# Autodesk Inventor assembly: Window_Cabinet
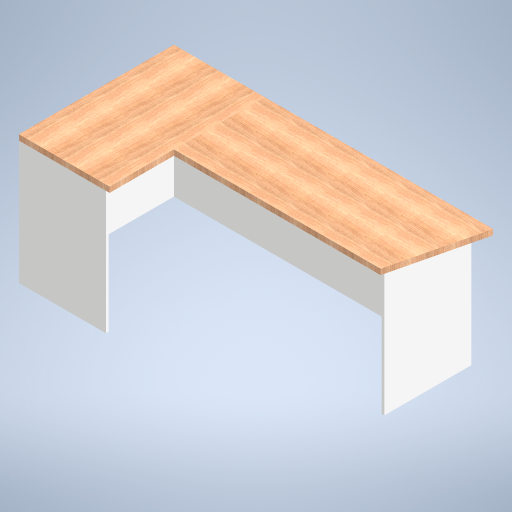
[picture p0: Inventor's stored thumbnail of the model, 512x512]
Saved by Autodesk Inventor 2024 (Build 280153000, 153)
## iProperties
Created: 2023-05-06
Part Number: Window_Cabinet
Document SubType Name: Assembly
Designer: Tom
Author: Tom
## Documents named in this file (6)
- C:\Users\Tom\Documents\Tom_Levers_Public_Git_Repository\Inventor\Mobility\Window_Cabinet\Window_Cabinet.iam
- C:\Users\Tom\Documents\Tom_Levers_Public_Git_Repository\Inventor\Mobility\Window_Cabinet\Plywood--0.75_x_34_x_88_in.ipt
- C:\Users\Tom\Documents\Tom_Levers_Public_Git_Repository\Inventor\Mobility\Window_Cabinet\Plywood--0.75_x_34_x_42_in.ipt
- C:\Users\Tom\Documents\Tom_Levers_Public_Git_Repository\Inventor\Mobility\Window_Cabinet\Plywood--0.75_x_34_x_23.25_in.ipt
- C:\Users\Tom\Documents\Tom_Levers_Public_Git_Repository\Inventor\Mobility\Window_Cabinet\Butcher_Block--1.5_x_25_x_42.75_in.ipt
- C:\Users\Tom\Documents\Tom_Levers_Public_Git_Repository\Inventor\Mobility\Window_Cabinet\Butcher_Block--1.5_x_25_x_64_in--Cut.ipt
## Components (6 placed, 5 different names)
1. Plywood--0.75_x_34_x_88_in:1 — Mate:1, Flush:1, Flush:2, Flush:7, Mate:4, Mate:5, Flush:9, Mate:7, Flush:10, Flush:11
2. Plywood--0.75_x_34_x_42_in:1 — Mate:1, Flush:1, Flush:2, Mate:3, Flush:5, Flush:6, Flush:8
3. Plywood--0.75_x_34_x_23.25_in:2 — Mate:3, Flush:5, Flush:6
4. Butcher_Block--1.5_x_25_x_42.75_in:1 — Flush:7, Mate:4, Flush:8, Mate:6
5. Butcher_Block--1.5_x_25_x_64_in--Cut:1 — Mate:5, Mate:6, Flush:9
6. Plywood--0.75_x_34_x_23.25_in:3 — Mate:7, Flush:10, Flush:11
## Relationships (15: Flush 9, Mate 6)
- Mate:1: Plywood--0.75_x_34_x_88_in:1 ↔ Plywood--0.75_x_34_x_42_in:1
- Flush:1: Plywood--0.75_x_34_x_88_in:1 ↔ Plywood--0.75_x_34_x_42_in:1
- Flush:2: Plywood--0.75_x_34_x_88_in:1 ↔ Plywood--0.75_x_34_x_42_in:1
- Mate:3: Plywood--0.75_x_34_x_42_in:1 ↔ Plywood--0.75_x_34_x_23.25_in:2
- Flush:5: Plywood--0.75_x_34_x_42_in:1 ↔ Plywood--0.75_x_34_x_23.25_in:2
- Flush:6: Plywood--0.75_x_34_x_42_in:1 ↔ Plywood--0.75_x_34_x_23.25_in:2
- Flush:7: Plywood--0.75_x_34_x_88_in:1 ↔ Butcher_Block--1.5_x_25_x_42.75_in:1
- Mate:4: Plywood--0.75_x_34_x_88_in:1 ↔ Butcher_Block--1.5_x_25_x_42.75_in:1
- Flush:8: Plywood--0.75_x_34_x_42_in:1 ↔ Butcher_Block--1.5_x_25_x_42.75_in:1
- Mate:5: Plywood--0.75_x_34_x_88_in:1 ↔ Butcher_Block--1.5_x_25_x_64_in--Cut:1
- Mate:6: Butcher_Block--1.5_x_25_x_42.75_in:1 ↔ Butcher_Block--1.5_x_25_x_64_in--Cut:1
- Flush:9: Plywood--0.75_x_34_x_88_in:1 ↔ Butcher_Block--1.5_x_25_x_64_in--Cut:1
- Mate:7: Plywood--0.75_x_34_x_88_in:1 ↔ Plywood--0.75_x_34_x_23.25_in:3
- Flush:10: Plywood--0.75_x_34_x_88_in:1 ↔ Plywood--0.75_x_34_x_23.25_in:3
- Flush:11: Plywood--0.75_x_34_x_88_in:1 ↔ Plywood--0.75_x_34_x_23.25_in:3
